# Autodesk Inventor assembly: Montagem2
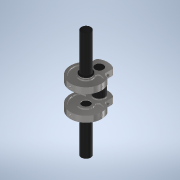
[picture p0: Inventor's stored thumbnail of the model, 180x180]
Saved by Autodesk Inventor 2021 (Build 250183000, 183)
## iProperties
Created: 2021-07-18
Part Number: Montagem2
Document SubType Name: Assembly
Designer: Giovanni
Author: Giovanni
## Documents named in this file (6)
- C:\Users\irineu\Documents\Inventor\MotorRadial7\Montagem2.iam
- C:\Users\irineu\Documents\Inventor\MotorRadial7\Peça15.ipt
- C:\Users\irineu\Documents\Inventor\MotorRadial7\Peça13.ipt
- C:\Users\irineu\Documents\Inventor\MotorRadial7\Peça12.ipt
- C:\Users\irineu\Documents\Inventor\MotorRadial7\Peça11.ipt
- C:\Users\irineu\Documents\Inventor\Content Center Files\R2021\pt-BR\DIN 913\DIN 913 - M8 x 25.ipt
## Components (17 placed, 5 different names)
1. Peça15:1 — Inserir:1, Inserir:4, Coincidente:2, Coincidente:4
2. Peça13:1 — Inserir:1, Inserir:2, Tangente:1, Tangente:2
3. Peça15:2 — Inserir:2, Coincidente:1, Inserir:3, Coincidente:3, Coincidente:5
4. Peça12:1 — Inserir:3, Alinhado:1, Tangente:4
5. Peça11:1 — Inserir:4, Tangente:3
6. DIN 913 M8 x 25:1 — Coincidente:2, Tangente:1
7. DIN 913 M8 x 25:2 — Coincidente:3, Tangente:2
8. DIN 913 M8 x 25:5
9. DIN 913 M8 x 25:6
10. DIN 913 M8 x 25:7
11. DIN 913 M8 x 25:8
12. DIN 913 M8 x 25:3 — Coincidente:4, Tangente:3
13. DIN 913 M8 x 25:4 — Coincidente:5, Tangente:4
14. DIN 913 M8 x 25:9
15. DIN 913 M8 x 25:10
16. DIN 913 M8 x 25:11
17. DIN 913 M8 x 25:12
## Component patterns: (3 elements, first: DIN 913 M8 x 25:1 + DIN 913 M8 x 25:2), (3 elements, first: DIN 913 M8 x 25:3 + DIN 913 M8 x 25:4)
## Relationships (14: Mate 5, Insert 4, Tangent 4, Flush 1)
- Inserir:1: Peça15:1 ↔ Peça13:1
- Inserir:2: Peça13:1 ↔ Peça15:2
- Coincidente:1 [Mate]: Peça15:2
- Inserir:3: Peça15:2 ↔ Peça12:1
- Alinhado:1 [Flush]: Peça12:1
- Inserir:4: Peça15:1 ↔ Peça11:1
- Coincidente:2 [Mate]: Peça15:1 ↔ DIN 913 M8 x 25:1
- Coincidente:3 [Mate]: Peça15:2 ↔ DIN 913 M8 x 25:2
- Tangente:1: Peça13:1 ↔ DIN 913 M8 x 25:1
- Tangente:2: Peça13:1 ↔ DIN 913 M8 x 25:2
- Coincidente:4 [Mate]: Peça15:1 ↔ DIN 913 M8 x 25:3
- Coincidente:5 [Mate]: Peça15:2 ↔ DIN 913 M8 x 25:4
- Tangente:3: Peça11:1 ↔ DIN 913 M8 x 25:3
- Tangente:4: Peça12:1 ↔ DIN 913 M8 x 25:4
